# Autodesk Inventor assembly: BallOnBeam
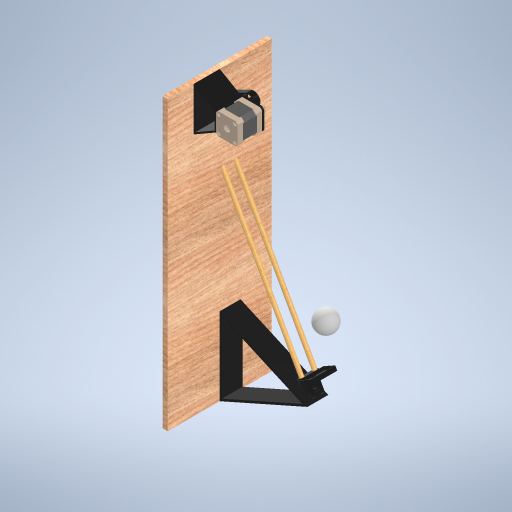
[picture p0: Inventor's stored thumbnail of the model, 512x512]
Saved by Autodesk Inventor 2023 (Build 270158000, 158)
## iProperties
Created: 2024-01-25
Part Number: BallOnBeam
Document SubType Name: Assembly
Designer: phili
Author: phili
## Documents named in this file (11)
- C:\Users\phili\FAUbox\Philipp\Bauprojekte\Ball_On_Beam\CAD\BallOnBeam.iam
- C:\Users\phili\FAUbox\Philipp\Bauprojekte\Ball_On_Beam\CAD\Bauteile\Grundfläche.ipt
- C:\Users\phili\FAUbox\Philipp\Bauprojekte\Ball_On_Beam\CAD\Bauteile\MotorHalterung.ipt
- C:\Users\phili\FAUbox\Philipp\Bauprojekte\Ball_On_Beam\CAD\Bauteile\nema17-stepping-motor-1.snapshot.1\Assem Stepper Motor.ipt
- C:\Users\phili\FAUbox\Philipp\Bauprojekte\Ball_On_Beam\CAD\Bauteile\Motoranker.ipt
- C:\Users\phili\FAUbox\Philipp\Bauprojekte\Ball_On_Beam\CAD\Bauteile\Hebel.ipt
- C:\Users\phili\FAUbox\Philipp\Bauprojekte\Ball_On_Beam\CAD\Bauteile\SensorArm.ipt
- C:\Users\phili\FAUbox\Philipp\Bauprojekte\Ball_On_Beam\CAD\Bauteile\ObenMotor.ipt
- C:\Users\phili\FAUbox\Philipp\Bauprojekte\Ball_On_Beam\CAD\Bauteile\Stab.ipt
- C:\Users\phili\FAUbox\Philipp\Bauprojekte\Ball_On_Beam\CAD\Bauteile\SensohalterMount.iam
- C:\Users\phili\FAUbox\Philipp\Bauprojekte\Ball_On_Beam\CAD\Bauteile\Ball.ipt
## Components (11 placed, 10 different names)
1. Grundfläche:1 — Passend:1, Fluchtend:1, Passend:28, Passend:29, Passend:32
2. MotorHalterung:1 — Passend:1, Fluchtend:1, Passend:3, Passend:4, Passend:5, Passend:6, Passend:28
3. Assem Stepper Motor:1 — Passend:3, Passend:4, Passend:5, Passend:7
4. Motoranker:1 — Passend:6, Passend:7, Passend:8, Passend:9, Winkel:1, Winkel:2
5. Hebel:1 — Passend:8, Passend:9, Passend:19, Passend:20, Winkel:2, Winkel:3
6. SensorArm:1 — Passend:29, Passend:30, Passend:31, Passend:32
7. ObenMotor:1 — Passend:19, Passend:20, Winkel:3, Passend:21, Passend:22, Passend:23, Passend:24
8. Stab:1 — Passend:23, Passend:24, Passend:26
9. Stab:2 — Passend:21, Passend:22, Passend:25, Passend:27
10. SensohalterMount:1 [sub-assembly] — Passend:25, Passend:26, Passend:27, Passend:30, Passend:31
11. Ball:1
## Relationships (26: Mate 22, Angle 3, Flush 1)
- Passend:1 [Mate]: Grundfläche:1 ↔ MotorHalterung:1
- Fluchtend:1 [Flush] (100 mm): Grundfläche:1 ↔ MotorHalterung:1
- Passend:3 [Mate]: MotorHalterung:1 ↔ Assem Stepper Motor:1
- Passend:4 [Mate]: MotorHalterung:1 ↔ Assem Stepper Motor:1
- Passend:5 [Mate]: MotorHalterung:1 ↔ Assem Stepper Motor:1
- Passend:6 [Mate]: MotorHalterung:1 ↔ Motoranker:1
- Passend:7 [Mate]: Assem Stepper Motor:1 ↔ Motoranker:1
- Passend:8 [Mate]: Motoranker:1 ↔ Hebel:1
- Passend:9 [Mate]: Motoranker:1 ↔ Hebel:1
- Passend:19 [Mate]: Hebel:1 ↔ ObenMotor:1
- Passend:20 [Mate]: Hebel:1 ↔ ObenMotor:1
- Winkel:1 [Angle] (90 deg): Motoranker:1
- Winkel:2 [Angle] (-90 deg): Motoranker:1 ↔ Hebel:1
- Winkel:3 [Angle] (90 deg): Hebel:1 ↔ ObenMotor:1
- Passend:21 [Mate]: ObenMotor:1 ↔ Stab:2
- Passend:22 [Mate]: ObenMotor:1 ↔ Stab:2
- Passend:23 [Mate]: ObenMotor:1 ↔ Stab:1
- Passend:24 [Mate]: ObenMotor:1 ↔ Stab:1
- Passend:25 [Mate]: Stab:2 ↔ SensohalterMount:1
- Passend:26 [Mate]: Stab:1 ↔ SensohalterMount:1
- Passend:27 [Mate]: Stab:2 ↔ SensohalterMount:1
- Passend:28 [Mate]: Grundfläche:1 ↔ MotorHalterung:1
- Passend:29 [Mate]: Grundfläche:1 ↔ SensorArm:1
- Passend:30 [Mate]: SensorArm:1 ↔ SensohalterMount:1
- Passend:31 [Mate]: SensorArm:1 ↔ SensohalterMount:1
- Passend:32 [Mate]: Grundfläche:1 ↔ SensorArm:1
